# Autodesk Inventor assembly: LegAssembly
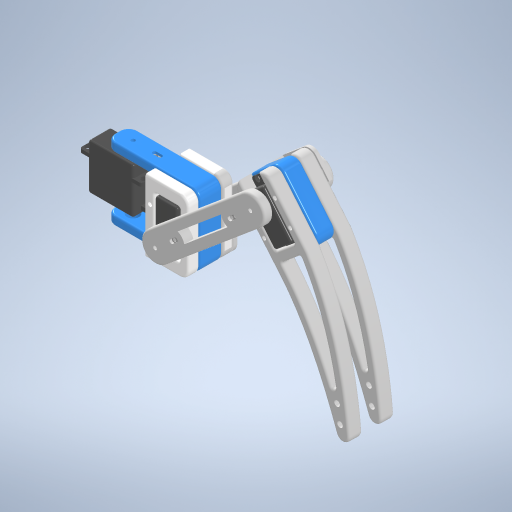
[picture p0: Inventor's stored thumbnail of the model, 512x512]
Saved by Autodesk Inventor 2024 (Build 280153000, 153)
## iProperties
Created: 2025-12-19
Part Number: LegAssembly
Document SubType Name: Assembly
Designer: Liam
Mass: 308.194 g
Surface Area: 1190.38 cm^2
Volume: 308.194 cm^3
Density: 1 g/cm^3
Author: Liam
## Documents named in this file (12)
- C:\Users\Liam\OneDrive\Documents\Inventor\Hexapod\LegAssembly.iam
- C:\Users\Liam\OneDrive\Documents\Inventor\Hexapod\Servo40KgRough.ipt
- C:\Users\Liam\OneDrive\Documents\Inventor\Hexapod\ServoMount.ipt
- C:\Users\Liam\OneDrive\Documents\Inventor\Hexapod\TibiaLeft.ipt
- C:\Users\Liam\OneDrive\Documents\Inventor\Hexapod\Horn.ipt
- C:\Users\Liam\OneDrive\Documents\Inventor\Hexapod\FemurHornSide.ipt
- C:\Users\Liam\OneDrive\Documents\Inventor\Hexapod\TibiaRight.ipt
- C:\Users\Liam\OneDrive\Documents\Inventor\Hexapod\FemurPivotSide.ipt
- C:\Users\Liam\OneDrive\Documents\Inventor\Hexapod\CoxaHornSide.ipt
- C:\Users\Liam\OneDrive\Documents\Inventor\Hexapod\CoxaPivotSide.ipt
- C:\Users\Liam\OneDrive\Documents\Inventor\Hexapod\CoxaLeft.ipt
- C:\Users\Liam\OneDrive\Documents\Inventor\Hexapod\CoxaRight.ipt
## Components (15 placed, 11 different names)
1. Servo40KgRough:1 — Knee Servo -> Knee Horn, Knee Servo -> Knee Mount
2. ServoMount:1 — Knee Servo -> Knee Mount, Knee Mount -> Tibia Left, Knee Mount -> Tibia Right
3. TibiaLeft:2 — Knee Mount -> Tibia Left
4. Horn:1 — Knee Servo -> Knee Horn, Knee Horn -> Femur Left
5. FemurHornSide:1 — Knee Horn -> Femur Left, Femur Horn -> Femur Left
6. TibiaRight:1 — Knee Mount -> Tibia Right, Tibia Right -> Femur Right
7. FemurPivotSide:1 — Coxa Right -> Femur Right, Tibia Right -> Femur Right
8. CoxaHornSide:1 — Coxa Horn -> Coxa Top, Coxa Bottom -> Coxa Right, Rigid:16
9. Servo40KgRough:2 — Femur Servo -> Femur Horn, Rigid:16, Rigid:17
10. Horn:2 — Femur Servo -> Femur Horn, Femur Horn -> Femur Left
11. CoxaLeft:1 — Coxa Botttom -> Coxa Left
12. CoxaRight:1 — Coxa Right -> Femur Right, Coxa Bottom -> Coxa Right
13. Servo40KgRough:3 — Coxa Servo -> Coxa Horn
14. Horn:3 — Coxa Servo -> Coxa Horn, Coxa Horn -> Coxa Top
15. CoxaPivotSide:1 — Coxa Botttom -> Coxa Left, Rigid:17
## Relationships (15: WeldJoint 10, RevoluteJoint 5)
- Knee Servo -> Knee Horn [RevoluteJoint]: Servo40KgRough:1 ↔ Horn:1
- Knee Servo -> Knee Mount [WeldJoint]: Servo40KgRough:1 ↔ ServoMount:1
- Knee Mount -> Tibia Left [WeldJoint]: ServoMount:1 ↔ TibiaLeft:2
- Knee Horn -> Femur Left [WeldJoint]: Horn:1 ↔ FemurHornSide:1
- Knee Mount -> Tibia Right [WeldJoint]: ServoMount:1 ↔ TibiaRight:1
- Femur Servo -> Femur Horn [RevoluteJoint]: Servo40KgRough:2 ↔ Horn:2
- Femur Horn -> Femur Left [WeldJoint]: FemurHornSide:1 ↔ Horn:2
- Coxa Servo -> Coxa Horn [RevoluteJoint]: Servo40KgRough:3 ↔ Horn:3
- Coxa Right -> Femur Right [RevoluteJoint]: FemurPivotSide:1 ↔ CoxaRight:1
- Coxa Horn -> Coxa Top [WeldJoint]: CoxaHornSide:1 ↔ Horn:3
- Coxa Botttom -> Coxa Left [WeldJoint]: CoxaLeft:1 ↔ CoxaPivotSide:1
- Coxa Bottom -> Coxa Right [WeldJoint]: CoxaHornSide:1 ↔ CoxaRight:1
- Tibia Right -> Femur Right [RevoluteJoint]: TibiaRight:1 ↔ FemurPivotSide:1
- Rigid:16 [WeldJoint]: CoxaHornSide:1 ↔ Servo40KgRough:2
- Rigid:17 [WeldJoint]: Servo40KgRough:2 ↔ CoxaPivotSide:1
## Named parameters: KneeJoint = 80 deg, TrochanterJoint = 45 deg, CoxaJoint = 0 deg
